# Autodesk Inventor assembly: robot_new
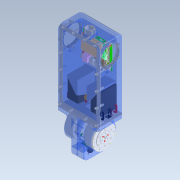
[picture p0: Inventor's stored thumbnail of the model, 180x180]
Saved by Autodesk Inventor 2020 (Build 240168000, 168)
## iProperties
Created: 2021-02-21
Part Number: robot_new
Document SubType Name: Assembly
Designer: DELL
Author: DELL
## Documents named in this file (8)
- F:\SoftRobot2.0\FlexipodHardware2.0\FlexipodHardware\Flexipod2.0\robot_2021_2_17\robot_new.0003.iam
- F:\SoftRobot2.0\FlexipodHardware2.0\FlexipodHardware\Flexipod2.0\robot_2021_2_17\back_hip_new.ipt
- F:\SoftRobot2.0\FlexipodHardware2.0\FlexipodHardware\Flexipod2.0\RMD_X6_stator.ipt
- F:\SoftRobot2.0\FlexipodHardware2.0\FlexipodHardware\Flexipod2.0\RMD_X6_rotor.ipt
- F:\SoftRobot2.0\FlexipodHardware2.0\FlexipodHardware\Flexipod2.0\Arducam Camera.ipt
- F:\SoftRobot2.0\FlexipodHardware2.0\FlexipodHardware\Flexipod2.0\robot_2021_2_17\body_soft.ipt
- F:\SoftRobot2.0\FlexipodHardware2.0\FlexipodHardware\Flexipod2.0\Jetson nano v2- Inventor\Jetson_Nano_Dev_Kit_3D_b01.iam
- F:\SoftRobot2.0\FlexipodHardware2.0\FlexipodHardware\Flexipod2.0\battery_6s_1550_ovonic.ipt
## Components (10 placed, 7 different names)
1. back_hip_new:1 — Flush:3, Flush:2, Mate:3, Mate:4, Mate:5, Mate:8, Mate:12, Mate:13, Mate:14, Mate:23, Flush:5, Flush:6, Mate:35, Mate:36, Mate:37
2. RMD_X6_stator:1 — Mate:1, Flush:1, Mate:3, Mate:4, Mate:5
3. RMD_X6_rotor:1 — Mate:1, Flush:1
4. Arducam Camera:1 — Mate:12, Mate:13, Mate:14
5. body_soft:1 — Mate:23, Flush:5, Flush:6, Mate:25, Mate:26, Mate:27, Mate:28, Mate:29, Mate:30, Mate:31, Mate:32, Mate:33
6. Jetson_Nano_Dev_Kit_3D_b01:1 [sub-assembly] — Mate:25, Mate:26, Mate:27
7. battery_6s_1550_ovonic:1 — Mate:28, Mate:29, Mate:30
8. battery_6s_1550_ovonic:2 — Mate:31, Mate:32, Mate:33
9. RMD_X6_stator:3 — Mate:35, Mate:36, Mate:37
10. RMD_X6_rotor:3
## Relationships (28: Mate 22, Flush 6)
- Mate:1: RMD_X6_stator:1 ↔ RMD_X6_rotor:1
- Flush:1 (-0.5 mm): RMD_X6_stator:1 ↔ RMD_X6_rotor:1
- Flush:3: back_hip_new:1
- Flush:2: back_hip_new:1
- Mate:3: back_hip_new:1 ↔ RMD_X6_stator:1
- Mate:4: back_hip_new:1 ↔ RMD_X6_stator:1
- Mate:5: back_hip_new:1 ↔ RMD_X6_stator:1
- Mate:8: back_hip_new:1
- Mate:12: back_hip_new:1 ↔ Arducam Camera:1
- Mate:13: back_hip_new:1 ↔ Arducam Camera:1
- Mate:14: back_hip_new:1 ↔ Arducam Camera:1
- Mate:23: back_hip_new:1 ↔ body_soft:1
- Flush:5: back_hip_new:1 ↔ body_soft:1
- Flush:6: back_hip_new:1 ↔ body_soft:1
- Mate:25: body_soft:1 ↔ Jetson_Nano_Dev_Kit_3D_b01:1
- Mate:26: body_soft:1 ↔ Jetson_Nano_Dev_Kit_3D_b01:1
- Mate:27: body_soft:1 ↔ Jetson_Nano_Dev_Kit_3D_b01:1
- Mate:28: body_soft:1 ↔ battery_6s_1550_ovonic:1
- Mate:29: body_soft:1 ↔ battery_6s_1550_ovonic:1
- Mate:30: body_soft:1 ↔ battery_6s_1550_ovonic:1
- Mate:31: body_soft:1 ↔ battery_6s_1550_ovonic:2
- Mate:32: body_soft:1 ↔ battery_6s_1550_ovonic:2
- Mate:33: body_soft:1 ↔ battery_6s_1550_ovonic:2
- [Mate]: RMD_X6_stator:3 ↔ RMD_X6_rotor:3
- [Flush] (-0.5 mm): RMD_X6_stator:3 ↔ RMD_X6_rotor:3
- Mate:35: back_hip_new:1 ↔ RMD_X6_stator:3
- Mate:36: back_hip_new:1 ↔ RMD_X6_stator:3
- Mate:37: back_hip_new:1 ↔ RMD_X6_stator:3
## Named parameters: d39_d24 = 0 mm, d40_d25 = -0.5 mm
